# Autodesk Inventor assembly: !Tower
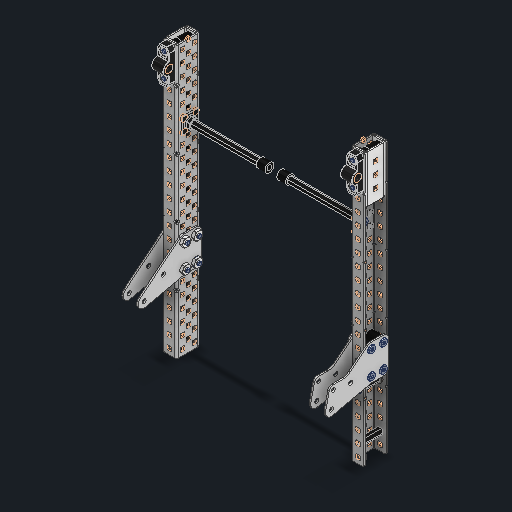
[picture p0: Inventor's stored thumbnail of the model, 512x512]
Saved by Autodesk Inventor 2025.1 (Build 291241000, 241)
## iProperties
Created: 2024-10-20
Part Number: !Tower
Document SubType Name: Assembly
Designer: Averey Ku
Author: Averey Ku
## Documents named in this file (3)
- C:\Users\avere\VEX\High Stakes\CAD\V2\Tower\!Tower.iam
- C:\Users\avere\VEX\High Stakes\CAD\V2\Tower\Left Structure.iam
- C:\Users\avere\VEX\High Stakes\CAD\V2\Tower\Right Structure\Right Structure.iam
## Components (2 placed, 2 different names)
1. Left Structure:1 [sub-assembly] — Mate:3, Flush:1, Insert:1, Mate:4
2. Right Structure:1 [sub-assembly] — Insert:1, Mate:4
## Relationships (5: Mate 3, Flush 1, Insert 1)
- [Mate]: Left Structure:1 ↔ Right Structure:1
- Mate:3 (-146.05 mm): Left Structure:1
- Flush:1 (-12.7 mm): Left Structure:1
- Insert:1 (12.7362 mm): Left Structure:1 ↔ Right Structure:1
- Mate:4: Left Structure:1 ↔ Right Structure:1
